# Autodesk Inventor assembly: Connessione B
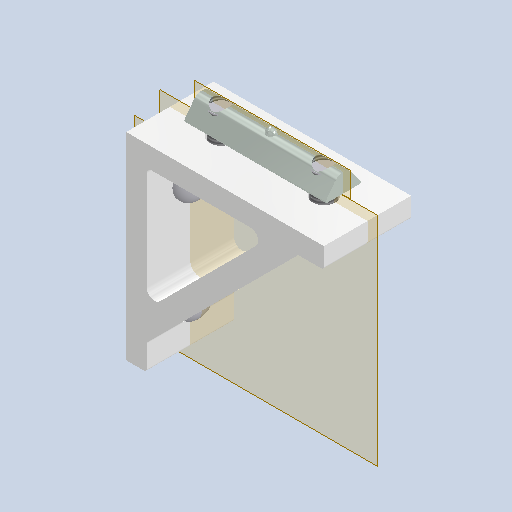
[picture p0: Inventor's stored thumbnail of the model, 512x512]
Saved by Autodesk Inventor 2022 (Build 260153000, 153)
## iProperties
Created: 2022-01-26
Part Number: Connessione B
Document SubType Name: Assembly
Designer: matte
Author: matte
## Documents named in this file (4)
- C:\Users\matte\Documents\GitHub\MDM-CyberOrto-CAD\Assiemi\Connessione B.iam
- C:\Users\matte\Documents\GitHub\MDM-CyberOrto-CAD\Parker components\03-Brackets_Gussets_Plates\09-Machined Gussets\20-102.ipt
- C:\Users\matte\Documents\GitHub\MDM-CyberOrto-CAD\Parker components\02-Fasteners\10-Standard T-Nuts\20-050.ipt
- C:\Users\matte\Documents\GitHub\MDM-CyberOrto-CAD\Parker components\02-Fasteners\16-Screws\01-Metric Screws\01-Button Head\24-118-8.ipt
## Components (7 placed, 3 different names)
1. 20-102:1
2. 20-050:1
3. 20-050:2
4. 24-118-8:1
5. 24-118-8:2
6. 24-118-8:3
7. 24-118-8:4
## Relationships (12: Mate 12)
- [Mate]: 20-102:1 ↔ 20-050:1
- [Mate]: 20-102:1 ↔ 20-050:1
- [Mate]: 20-102:1 ↔ 20-050:2
- [Mate]: 20-102:1 ↔ 20-050:2
- [Mate]: 20-102:1 ↔ 24-118-8:1
- [Mate]: 20-102:1 ↔ 24-118-8:1
- [Mate]: 20-102:1 ↔ 24-118-8:2
- [Mate]: 20-102:1 ↔ 24-118-8:2
- [Mate]: 20-102:1 ↔ 24-118-8:3
- [Mate]: 20-102:1 ↔ 24-118-8:3
- [Mate]: 20-102:1 ↔ 24-118-8:4
- [Mate]: 20-102:1 ↔ 24-118-8:4
